# Autodesk Inventor assembly: Avionics
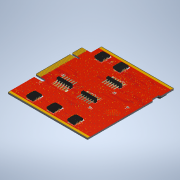
[picture p0: Inventor's stored thumbnail of the model, 180x180]
Saved by Autodesk Inventor 2021 (Build 250183000, 183)
## iProperties
Created: 2020-10-20
Part Number: Avionics
Document SubType Name: Assembly
Designer: Bradley
Author: Bradley
## Documents named in this file (35)
- C:\Users\Bradley\Documents\GitHub\CougSat1-Hardware\CougSat1-AvionicBoard\CADModel\Native\Avionics.iam
- C:\Users\Bradley\Documents\GitHub\CougSat1-Hardware\CougSat1-AvionicBoard\CADModel\Native\Avionics_PCB.ipt
- C:\Users\Bradley\Documents\GitHub\Resources\SupplierDocuments\04 - Connectors SMT\04-0001\04-0001.iam
- C:\Users\Bradley\Documents\GitHub\Resources\SupplierDocuments\04 - Connectors SMT\04-0008\04-0008.iam
- C:\Users\Bradley\Documents\GitHub\Resources\SupplierDocuments\21 - Resistor 1608\21-0000\21-0000.ipt
- C:\Users\Bradley\Documents\GitHub\Resources\SupplierDocuments\36 - Ferrite\36-152A\36-152A.ipt
- C:\Users\Bradley\Documents\GitHub\Resources\SupplierDocuments\11 - Capacitor Ceramic 1608\11-105A\11-105A.ipt
- C:\Users\Bradley\Documents\GitHub\Resources\SupplierDocuments\21 - Resistor 1608\21-1001\21-1001.ipt
- C:\Users\Bradley\Documents\GitHub\Resources\SupplierDocuments\16 - Capacitor Tantalum SMT\16-475A\16-475A.ipt
- C:\Users\Bradley\Documents\GitHub\Resources\SupplierDocuments\11 - Capacitor Ceramic 1608\11-682A\11-682A.ipt
- C:\Users\Bradley\Documents\GitHub\Resources\SupplierDocuments\40 - Crystal SMT\40-805A\40-805A.ipt
- C:\Users\Bradley\Documents\GitHub\Resources\SupplierDocuments\11 - Capacitor Ceramic 1608\11-106A\11-106A.ipt
- C:\Users\Bradley\Documents\GitHub\Resources\SupplierDocuments\21 - Resistor 1608\21-1002\21-1002.ipt
- C:\Users\Bradley\Documents\GitHub\Resources\SupplierDocuments\26 - Resistor Misc\26-0001\26-0001.ipt
- C:\Users\Bradley\Documents\GitHub\Resources\SupplierDocuments\26 - Resistor Misc\26-0008\26-0008.ipt
- C:\Users\Bradley\Documents\GitHub\Resources\SupplierDocuments\11 - Capacitor Ceramic 1608\11-103A\11-103A.ipt
- C:\Users\Bradley\Documents\GitHub\Resources\SupplierDocuments\11 - Capacitor Ceramic 1608\11-100A\11-100A.ipt
- C:\Users\Bradley\Documents\GitHub\Resources\SupplierDocuments\11 - Capacitor Ceramic 1608\11-150A\11-150A.ipt
- C:\Users\Bradley\Documents\GitHub\Resources\SupplierDocuments\26 - Resistor Misc\26-0006\26-0006.ipt
- C:\Users\Bradley\Documents\GitHub\Resources\SupplierDocuments\40 - Crystal SMT\40-323A\40-323A.ipt
- C:\Users\Bradley\Documents\GitHub\Resources\SupplierDocuments\31 - Inductor 1608\31-330A\31-330A.ipt
- C:\Users\Bradley\Documents\GitHub\Resources\SupplierDocuments\16 - Capacitor Tantalum SMT\16-476A\16-476A.ipt
- C:\Users\Bradley\Documents\GitHub\Resources\SupplierDocuments\21 - Resistor 1608\21-0.05\21-0.05.ipt
- C:\Users\Bradley\Documents\GitHub\Resources\SupplierDocuments\11 - Capacitor Ceramic 1608\11-104A\11-104A.ipt
- C:\Users\Bradley\Documents\GitHub\Resources\SupplierDocuments\27 - Conversion IC\27-0003\27-0003.ipt
- C:\Users\Bradley\Documents\GitHub\Resources\SupplierDocuments\08 - Amplifier (excluding RF)\08-0002\08-0002.ipt
- C:\Users\Bradley\Documents\GitHub\Resources\SupplierDocuments\63 - LED SMT\63-0004\63-0004.ipt
- C:\Users\Bradley\Documents\GitHub\Resources\SupplierDocuments\63 - LED SMT\63-0001\63-0001.ipt
- C:\Users\Bradley\Documents\GitHub\Resources\SupplierDocuments\04 - Connectors SMT\04-0005\04-0005.ipt
- C:\Users\Bradley\Documents\GitHub\Resources\SupplierDocuments\08 - Amplifier (excluding RF)\08-0004\08-0004.ipt
- C:\Users\Bradley\Documents\GitHub\Resources\SupplierDocuments\29 - Memory\29-0001\29-0001.ipt
- C:\Users\Bradley\Documents\GitHub\Resources\SupplierDocuments\61 - µController (and CLPD, FPGA,  etc.)\61-0002\61-0002.ipt
- C:\Users\Bradley\Documents\GitHub\Resources\SupplierDocuments\04 - Connectors SMT\04-0004\04-0004.ipt
- C:\Users\Bradley\Documents\GitHub\Resources\SupplierDocuments\09 - Communication IC\09-0001\09-0001.ipt
- C:\Users\Bradley\Documents\GitHub\Resources\SupplierDocuments\65 - RF\65-0001\65-0001.ipt
## Components (205 placed, 34 different names)
1. 65-0001:1 — Mate:483, Mate:484, Flush:131
2. 09-0001:8 — Mate:469, Mate:482, Flush:130
3. 09-0001:7 — Mate:470, Mate:481, Flush:129
4. 09-0001:6 — Mate:471, Mate:480, Flush:128
5. 09-0001:5 — Mate:472, Mate:479, Flush:127
6. 09-0001:4 — Mate:473, Flush:125, Flush:126
7. 09-0001:3 — Mate:474, Flush:123, Flush:124
8. 09-0001:2 — Mate:475, Flush:122, Mate:478
9. 09-0001:1 — Mate:476, Flush:121, Mate:477
10. 04-0004:3 — Mate:463, Mate:468, Flush:120
11. 04-0004:2 — Mate:464, Flush:119, Mate:467
12. 04-0004:1 — Mate:465, Flush:118, Mate:466
13. 61-0002:3 — Mate:461, Flush:117, Mate:462
14. 61-0002:2 — Mate:460, Flush:115, Flush:116
15. 61-0002:1 — Mate:459, Flush:113, Flush:114
16. 29-0001:2 — Mate:458, Flush:111, Flush:112
17. 29-0001:1 — Mate:457, Flush:109, Flush:110
18. 08-0004:3 — Mate:456, Flush:107, Flush:108
19. 08-0004:2 — Mate:455, Flush:105, Flush:106
20. 08-0004:1 — Mate:454, Flush:103, Flush:104
21. 04-0005:4 — Mate:442, Mate:452, Mate:453
22. 04-0005:3 — Mate:443, Mate:450, Mate:451
23. 04-0005:2 — Mate:444, Mate:448, Mate:449
24. 04-0005:1 — Mate:445, Mate:446, Mate:447
25. 63-0001:3 — Mate:438, Mate:441, Flush:102
26. 63-0001:2 — Mate:434, Mate:440, Flush:101
27. 63-0001:1 — Mate:433, Mate:439, Flush:100
28. 63-0004:1 — Mate:432, Mate:436, Mate:437
29. 08-0002:4 — Mate:429, Mate:431, Flush:99
30. 08-0002:3 — Mate:428, Mate:430, Flush:98
31. 08-0002:2 — Mate:427, Flush:96, Flush:97
32. 08-0002:1 — Mate:426, Flush:94, Flush:95
33. 27-0003:3 — Mate:423, Mate:425, Flush:93
34. 27-0003:2 — Mate:422, Flush:91, Flush:92
35. 27-0003:1 — Mate:421, Mate:424, Flush:90
36. 11-104A:59 — Mate:299, Mate:419, Mate:420
37. 11-104A:58 — Mate:301, Mate:417, Mate:418
38. 11-104A:57 — Mate:302, Mate:416, Flush:89
39. 11-104A:56 — Mate:305, Mate:415, Flush:88
40. 11-104A:55 — Mate:306, Mate:413, Mate:414
41. 11-104A:54 — Mate:309, Mate:411, Mate:412
42. 11-104A:53 — Mate:312, Mate:410, Flush:87
43. 11-104A:52 — Mate:313, Mate:409, Flush:86
44. 11-104A:51 — Mate:314, Mate:407, Mate:408
45. 11-104A:50 — Mate:317, Mate:405, Mate:406
46. 11-104A:49 — Mate:318, Mate:403, Mate:404
47. 11-104A:48 — Mate:322, Mate:401, Mate:402
48. 11-104A:47 — Mate:323, Mate:399, Mate:400
49. 11-104A:46 — Mate:324, Mate:398, Flush:85
50. 11-104A:45 — Mate:327, Mate:396, Mate:397
51. 11-104A:44 — Mate:328, Mate:394, Mate:395
52. 11-104A:43 — Mate:331, Mate:392, Mate:393
53. 11-104A:42 — Mate:294, Mate:391, Flush:84
54. 11-104A:41 — Mate:295, Mate:389, Mate:390
55. 11-104A:40 — Mate:296, Mate:388, Flush:83
56. 11-104A:39 — Mate:297, Mate:387, Flush:82
57. 11-104A:38 — Mate:298, Mate:386, Flush:81
58. 11-104A:37 — Mate:300, Mate:384, Mate:385
59. 11-104A:36 — Mate:303, Mate:383, Flush:80
60. 11-104A:35 — Mate:304, Mate:381, Mate:382
61. 11-104A:34 — Mate:307, Mate:380, Flush:79
62. 11-104A:33 — Mate:308, Mate:378, Mate:379
63. 11-104A:32 — Mate:310, Mate:377, Flush:78
64. 11-104A:31 — Mate:311, Mate:376, Flush:77
65. 11-104A:30 — Mate:315, Mate:375, Flush:76
66. 11-104A:29 — Mate:316, Mate:373, Mate:374
67. 11-104A:28 — Mate:319, Mate:372, Flush:75
68. 11-104A:27 — Mate:320, Mate:370, Mate:371
69. 11-104A:26 — Mate:321, Mate:369, Flush:74
70. 11-104A:25 — Mate:325, Mate:368, Flush:73
71. 11-104A:24 — Mate:326, Mate:367, Flush:72
72. 11-104A:23 — Mate:329, Mate:365, Mate:366
73. 11-104A:22 — Mate:330, Mate:364, Flush:71
74. 11-104A:21 — Mate:293, Mate:362, Mate:363
75. 11-104A:20 — Mate:291, Mate:360, Mate:361
76. 11-104A:19 — Mate:292, Mate:359, Flush:70
77. 11-104A:18 — Mate:290, Mate:358, Flush:69
78. 11-104A:17 — Mate:289, Mate:356, Mate:357
79. 11-104A:16 — Mate:288, Mate:355, Flush:68
80. 11-104A:15 — Mate:287, Mate:353, Mate:354
81. 11-104A:14 — Mate:286, Mate:351, Mate:352
82. 11-104A:13 — Mate:285, Mate:350, Flush:67
83. 11-104A:12 — Mate:284, Mate:349, Flush:66
84. 11-104A:11 — Mate:283, Mate:347, Mate:348
85. 11-104A:10 — Mate:282, Mate:346, Flush:65
86. 11-104A:9 — Mate:281, Mate:344, Mate:345
87. 11-104A:8 — Mate:280, Mate:343, Flush:64
88. 11-104A:7 — Mate:279, Mate:341, Mate:342
89. 11-104A:6 — Mate:278, Mate:340, Flush:63
90. 11-104A:5 — Mate:277, Mate:338, Mate:339
91. 11-104A:4 — Mate:276, Mate:336, Mate:337
92. 11-104A:3 — Mate:275, Mate:335, Flush:62
93. 11-104A:2 — Mate:274, Mate:334, Flush:61
94. 11-104A:1 — Mate:273, Mate:332, Mate:333
95. 21-0.05:3 — Mate:269, Mate:272, Flush:60
96. 21-0.05:2 — Mate:268, Mate:271, Flush:59
97. 21-0.05:1 — Mate:267, Mate:270, Flush:58
98. 16-476A:1 — Mate:264, Mate:265, Mate:266
99. 31-330A:1 — Mate:262, Mate:263, Flush:57
100. 40-323A:6 — Mate:251, Mate:260, Mate:261
101. 40-323A:5 — Mate:250, Mate:258, Mate:259
102. 40-323A:4 — Mate:249, Mate:256, Mate:257
103. 40-323A:3 — Mate:248, Mate:254, Mate:255
104. 40-323A:2 — Mate:247, Mate:253, Flush:56
105. 40-323A:1 — Mate:246, Mate:252, Flush:55
106. 26-0006:1 — Mate:243, Mate:244, Mate:245
107. 11-150A:12 — Mate:220, Mate:241, Mate:242
108. 11-150A:11 — Mate:219, Mate:239, Mate:240
109. 11-150A:10 — Mate:218, Mate:237, Mate:238
110. 11-150A:9 — Mate:217, Mate:235, Mate:236
111. 11-150A:8 — Mate:216, Mate:233, Mate:234
112. 11-150A:7 — Mate:215, Mate:231, Mate:232
113. 11-150A:6 — Mate:214, Mate:230, Flush:54
114. 11-150A:5 — Mate:213, Mate:229, Flush:53
115. 11-150A:4 — Mate:212, Mate:227, Mate:228
116. 11-150A:3 — Mate:211, Mate:225, Mate:226
117. 11-150A:2 — Mate:210, Mate:223, Mate:224
118. 11-150A:1 — Mate:209, Mate:221, Mate:222
119. 11-100A:6 — Mate:200, Mate:208, Flush:52
120. 11-100A:5 — Mate:199, Mate:206, Mate:207
121. 11-100A:4 — Mate:198, Mate:204, Mate:205
122. 11-100A:3 — Mate:197, Mate:203, Flush:51
123. 11-100A:2 — Mate:196, Mate:202, Flush:50
124. 11-100A:1 — Mate:195, Mate:201, Flush:49
125. 11-103A:3 — Mate:191, Mate:194, Flush:48
126. 11-103A:2 — Mate:190, Mate:193, Flush:47
127. 11-103A:1 — Mate:189, Mate:192, Flush:46
128. 26-0008:19 — Mate:160, Mate:187, Mate:188
129. 26-0008:18 — Mate:159, Mate:185, Mate:186
130. 26-0008:17 — Mate:158, Mate:184, Flush:45
131. 26-0008:16 — Mate:157, Mate:183, Flush:44
132. 26-0008:15 — Mate:156, Mate:181, Mate:182
133. 26-0008:14 — Mate:155, Mate:179, Mate:180
134. 26-0008:13 — Mate:154, Mate:178, Flush:43
135. 26-0008:12 — Mate:153, Mate:177, Flush:42
136. 26-0008:11 — Mate:152, Mate:175, Mate:176
137. 26-0008:10 — Mate:151, Mate:174, Flush:41
138. 26-0008:9 — Mate:150, Mate:173, Flush:40
139. 26-0008:8 — Mate:149, Mate:172, Flush:39
140. 26-0008:7 — Mate:148, Mate:171, Flush:38
141. 26-0008:6 — Mate:147, Mate:169, Mate:170
142. 26-0008:5 — Mate:146, Mate:167, Mate:168
143. 26-0008:4 — Mate:145, Mate:165, Mate:166
144. 26-0008:3 — Mate:144, Mate:163, Mate:164
145. 26-0008:2 — Mate:143, Mate:162, Flush:37
146. 26-0008:1 — Mate:142, Mate:161, Flush:36
147. 26-0001:3 — Mate:138, Mate:141, Flush:35
148. 26-0001:2 — Mate:137, Mate:140, Flush:34
149. 26-0001:1 — Mate:136, Mate:139, Flush:33
150. 21-1002:12 — Mate:116, Mate:133, Mate:134
151. 21-1002:11 — Mate:115, Mate:131, Mate:132
152. 21-1002:10 — Mate:114, Mate:130, Flush:31
153. 21-1002:9 — Mate:113, Mate:129, Flush:30
154. 21-1002:8 — Mate:112, Mate:128, Flush:29
155. 21-1002:7 — Mate:111, Mate:127, Flush:28
156. 21-1002:6 — Mate:110, Mate:126, Flush:27
157. 21-1002:5 — Mate:109, Mate:124, Mate:125
158. 21-1002:4 — Mate:108, Mate:123, Flush:26
159. 21-1002:3 — Mate:107, Mate:135, Flush:32
160. 21-1002:2 — Mate:106, Mate:119, Mate:120
161. 21-1002:1 — Mate:105, Mate:117, Mate:118
162. 11-106A:3 — Mate:98, Mate:103, Mate:104
163. 11-106A:2 — Mate:97, Mate:101, Mate:102
164. 11-106A:1 — Mate:96, Mate:99, Mate:100
165. 40-805A:3 — Mate:89, Mate:94, Mate:95
166. 40-805A:2 — Mate:90, Mate:93, Flush:25
167. 40-805A:1 — Mate:91, Mate:92, Flush:24
168. 11-682A:3 — Mate:85, Mate:88, Flush:23
169. 11-682A:2 — Mate:84, Mate:87, Flush:22
170. 11-682A:1 — Mate:83, Mate:86, Flush:21
171. 16-475A:2 — Mate:79, Mate:82, Flush:20
172. 16-475A:1 — Mate:78, Mate:80, Mate:81
173. 21-1001:11 — Mate:60, Mate:77, Flush:19
174. 21-1001:10 — Mate:59, Mate:76, Flush:18
175. 21-1001:9 — Mate:58, Mate:75, Flush:17
176. 21-1001:8 — Mate:57, Mate:73, Mate:74
177. 21-1001:7 — Mate:56, Mate:71, Mate:72
178. 21-1001:6 — Mate:55, Mate:69, Mate:70
179. 21-1001:5 — Mate:54, Mate:67, Mate:68
180. 21-1001:4 — Mate:53, Mate:65, Mate:66
181. 21-1001:3 — Mate:52, Mate:64, Flush:16
182. 21-1001:2 — Mate:51, Mate:62, Mate:63
183. 21-1001:1 — Mate:50, Mate:61, Flush:15
184. 11-105A:5 — Mate:41, Mate:48, Mate:49
185. 11-105A:4 — Mate:40, Mate:46, Mate:47
186. 11-105A:3 — Mate:39, Mate:44, Mate:45
187. 11-105A:2 — Mate:38, Mate:43, Flush:14
188. 11-105A:1 — Mate:37, Mate:42, Flush:13
189. 36-152A:2 — Mate:33, Mate:35, Mate:36
190. 36-152A:1 — Mate:32, Mate:34, Flush:12
191. 21-0000:7 — Mate:21, Mate:30, Mate:31
192. 21-0000:6 — Mate:20, Mate:29, Flush:11
193. 21-0000:5 — Mate:19, Mate:28, Flush:10
194. 21-0000:4 — Mate:18, Mate:26, Mate:27
195. 21-0000:3 — Mate:17, Mate:24, Mate:25
196. 21-0000:2 — Mate:16, Mate:23, Flush:9
197. 21-0000:1 — Mate:15, Mate:22, Flush:8
198. 04-0001:1 [sub-assembly] — Mate:1, Flush:1, Mate:8
199. 04-0001:2 [sub-assembly] — Mate:2, Flush:2, Mate:9
200. 04-0001:3 [sub-assembly] — Mate:3, Flush:3, Mate:10
201. 04-0001:4 [sub-assembly] — Mate:4, Flush:4, Mate:11
202. 04-0001:5 [sub-assembly] — Mate:5, Flush:5, Mate:12
203. 04-0001:6 [sub-assembly] — Mate:6, Flush:6, Mate:13
204. 04-0008:1 [sub-assembly] — Mate:7, Flush:7, Mate:14
205. Avionics_PCB:1 — Mate:1, Mate:2, Mate:3, Mate:4, Mate:5, Mate:6, Mate:7, Mate:15, Mate:16, Mate:17, Mate:18, Mate:19, Mate:20, Mate:21, Mate:32, Mate:33, Mate:37, Mate:38, Mate:39, Mate:40, Mate:41, Mate:50, Mate:51, Mate:52, Mate:53, Mate:54, Mate:55, Mate:56, Mate:57, Mate:58, Mate:59, Mate:60, Mate:78, Mate:79, Mate:83, Mate:84, Mate:85, Mate:89, Mate:90, Mate:91, Mate:96, Mate:97, Mate:98, Mate:105, Mate:106, Mate:107, Mate:108, Mate:109, Mate:110, Mate:111, Mate:112, Mate:113, Mate:114, Mate:115, Mate:116, Mate:136, Mate:137, Mate:138, Mate:142, Mate:143, Mate:144, Mate:145, Mate:146, Mate:147, Mate:148, Mate:149, Mate:150, Mate:151, Mate:152, Mate:153, Mate:154, Mate:155, Mate:156, Mate:157, Mate:158, Mate:159, Mate:160, Mate:189, Mate:190, Mate:191, Mate:195, Mate:196, Mate:197, Mate:198, Mate:199, Mate:200, Mate:209, Mate:210, Mate:211, Mate:212, Mate:213, Mate:214, Mate:215, Mate:216, Mate:217, Mate:218, Mate:219, Mate:220, Mate:243, Mate:246, Mate:247, Mate:248, Mate:249, Mate:250, Mate:251, Mate:262, Mate:264, Mate:267, Mate:268, Mate:269, Mate:273, Mate:274, Mate:275, Mate:276, Mate:277, Mate:278, Mate:279, Mate:280, Mate:281, Mate:282, Mate:283, Mate:284, Mate:285, Mate:286, Mate:287, Mate:288, Mate:289, Mate:290, Mate:291, Mate:292, Mate:293, Mate:294, Mate:295, Mate:296, Mate:297, Mate:298, Mate:299, Mate:300, Mate:301, Mate:302, Mate:303, Mate:304, Mate:305, Mate:306, Mate:307, Mate:308, Mate:309, Mate:310, Mate:311, Mate:312, Mate:313, Mate:314, Mate:315, Mate:316, Mate:317, Mate:318, Mate:319, Mate:320, Mate:321, Mate:322, Mate:323, Mate:324, Mate:325, Mate:326, Mate:327, Mate:328, Mate:329, Mate:330, Mate:331, Mate:421, Mate:422, Mate:423, Mate:426, Mate:427, Mate:428, Mate:429, Mate:432, Mate:433, Mate:434, Mate:438, Mate:442, Mate:443, Mate:444, Mate:445, Mate:454, Mate:455, Mate:456, Mate:457, Mate:458, Mate:459, Mate:460, Mate:461, Mate:463, Mate:464, Mate:465, Mate:469, Mate:470, Mate:471, Mate:472, Mate:473, Mate:474, Mate:475, Mate:476, Mate:483
## Relationships (612: Mate 481, Flush 131)
- Mate:1: 04-0001:1 ↔ Avionics_PCB:1
- Mate:2: 04-0001:2 ↔ Avionics_PCB:1
- Mate:3: 04-0001:3 ↔ Avionics_PCB:1
- Mate:4: 04-0001:4 ↔ Avionics_PCB:1
- Mate:5: 04-0001:5 ↔ Avionics_PCB:1
- Mate:6: 04-0001:6 ↔ Avionics_PCB:1
- Mate:7: 04-0008:1 ↔ Avionics_PCB:1
- Flush:1 (38 mm): 04-0001:1
- Flush:2 (38 mm): 04-0001:2
- Flush:3 (38 mm): 04-0001:3
- Flush:4 (-37.5 mm): 04-0001:4
- Flush:5 (-37.6 mm): 04-0001:5
- Mate:8 (25 mm): 04-0001:1
- Mate:9 (47.5 mm): 04-0001:2
- Mate:10 (70.5 mm): 04-0001:3
- Mate:11 (25 mm): 04-0001:4
- Mate:12 (45.5 mm): 04-0001:5
- Flush:6 (-84.2 mm): 04-0001:6
- Mate:13 (41 mm): 04-0001:6
- Flush:7 (12.1 mm): 04-0008:1
- Mate:14 (76.8 mm): 04-0008:1
- Mate:15: 21-0000:1 ↔ Avionics_PCB:1
- Mate:16: 21-0000:2 ↔ Avionics_PCB:1
- Mate:17: 21-0000:3 ↔ Avionics_PCB:1
- Mate:18: 21-0000:4 ↔ Avionics_PCB:1
- Mate:19: 21-0000:5 ↔ Avionics_PCB:1
- Mate:20: 21-0000:6 ↔ Avionics_PCB:1
- Mate:21: 21-0000:7 ↔ Avionics_PCB:1
- Mate:22 (9.5 mm): 21-0000:1
- Flush:8 (-12.5 mm): 21-0000:1
- Mate:23 (45 mm): 21-0000:2
- Flush:9 (-31.8 mm): 21-0000:2
- Mate:24 (-0.8 mm): 21-0000:3
- Mate:25 (54.4 mm): 21-0000:3
- Mate:26 (-6.5 mm): 21-0000:4
- Mate:27 (86.4 mm): 21-0000:4
- Mate:28 (34.2 mm): 21-0000:5
- Flush:10 (10.1 mm): 21-0000:5
- Mate:29 (52.4 mm): 21-0000:6
- Flush:11 (-30.8 mm): 21-0000:6
- Mate:30 (34.1 mm): 21-0000:7
- Mate:31 (26.8 mm): 21-0000:7
- Mate:32: 36-152A:1 ↔ Avionics_PCB:1
- Mate:33: 36-152A:2 ↔ Avionics_PCB:1
- Mate:34 (42.3 mm): 36-152A:1
- Flush:12 (-33.8 mm): 36-152A:1
- Mate:35 (15.9 mm): 36-152A:2
- Mate:36 (-19.3 mm): 36-152A:2
- Mate:37: 11-105A:1 ↔ Avionics_PCB:1
- Mate:38: 11-105A:2 ↔ Avionics_PCB:1
- Mate:39: 11-105A:3 ↔ Avionics_PCB:1
- Mate:40: 11-105A:4 ↔ Avionics_PCB:1
- Mate:41: 11-105A:5 ↔ Avionics_PCB:1
- Mate:42 (4.6 mm): 11-105A:1
- Flush:13 (-73.2 mm): 11-105A:1
- Mate:43 (-26.9 mm): 11-105A:2
- Flush:14 (-6.1 mm): 11-105A:2
- Mate:44 (8.6 mm): 11-105A:3
- Mate:45 (-29.3 mm): 11-105A:3
- Mate:46 (56.3 mm): 11-105A:4
- Mate:47 (32.7 mm): 11-105A:4
- Mate:48 (73.4 mm): 11-105A:5
- Mate:49 (32.8 mm): 11-105A:5
- Mate:50: 21-1001:1 ↔ Avionics_PCB:1
- Mate:51: 21-1001:2 ↔ Avionics_PCB:1
- Mate:52: 21-1001:3 ↔ Avionics_PCB:1
- Mate:53: 21-1001:4 ↔ Avionics_PCB:1
- Mate:54: 21-1001:5 ↔ Avionics_PCB:1
- Mate:55: 21-1001:6 ↔ Avionics_PCB:1
- Mate:56: 21-1001:7 ↔ Avionics_PCB:1
- Mate:57: 21-1001:8 ↔ Avionics_PCB:1
- Mate:58: 21-1001:9 ↔ Avionics_PCB:1
- Mate:59: 21-1001:10 ↔ Avionics_PCB:1
- Mate:60: 21-1001:11 ↔ Avionics_PCB:1
- Mate:61 (80.1 mm): 21-1001:1
- Flush:15 (-4 mm): 21-1001:1
- Mate:62 (17.6 mm): 21-1001:2
- Mate:63 (66.9 mm): 21-1001:2
- Mate:64 (67.5 mm): 21-1001:3
- Flush:16 (-19.9 mm): 21-1001:3
- Mate:65 (28.81 mm): 21-1001:4
- Mate:66 (56.41 mm): 21-1001:4
- Mate:67 (28.8 mm): 21-1001:5
- Mate:68 (54.7 mm): 21-1001:5
- Mate:69 (-1.99 mm): 21-1001:6
- Mate:70 (18.41 mm): 21-1001:6
- Mate:71 (25.3 mm): 21-1001:7
- Mate:72 (45.5 mm): 21-1001:7
- Mate:73 (-2.6 mm): 21-1001:8
- Mate:74 (45.6 mm): 21-1001:8
- Mate:75 (34.2 mm): 21-1001:9
- Flush:17 (14.7 mm): 21-1001:9
- Mate:76 (59 mm): 21-1001:10
- Flush:18 (-11.3 mm): 21-1001:10
- Mate:77 (59.1 mm): 21-1001:11
- Flush:19 (16.6 mm): 21-1001:11
- Mate:78: 16-475A:1 ↔ Avionics_PCB:1
- Mate:79: 16-475A:2 ↔ Avionics_PCB:1
- Mate:80 (40.2 mm): 16-475A:1
- Mate:81 (36.6 mm): 16-475A:1
- Mate:82 (13.7 mm): 16-475A:2
- Flush:20 (22.1 mm): 16-475A:2
- Mate:83: 11-682A:1 ↔ Avionics_PCB:1
- Mate:84: 11-682A:2 ↔ Avionics_PCB:1
- Mate:85: 11-682A:3 ↔ Avionics_PCB:1
- Mate:86 (27.3 mm): 11-682A:1
- Flush:21 (-35.6 mm): 11-682A:1
- Mate:87 (17.4 mm): 11-682A:2
- Flush:22 (-28.4 mm): 11-682A:2
- Mate:88 (27.2 mm): 11-682A:3
- Flush:23 (-17.9 mm): 11-682A:3
- Mate:89: 40-805A:3 ↔ Avionics_PCB:1
- Mate:90: 40-805A:2 ↔ Avionics_PCB:1
- Mate:91: 40-805A:1 ↔ Avionics_PCB:1
- Mate:92 (19.605 mm): 40-805A:1
- Flush:24 (-62.14 mm): 40-805A:1
- Mate:93 (-8.3 mm): 40-805A:2
- Flush:25 (-62.2 mm): 40-805A:2
- Mate:94 (27 mm): 40-805A:3
- Mate:95 (-17.8 mm): 40-805A:3
- Mate:96: 11-106A:1 ↔ Avionics_PCB:1
- Mate:97: 11-106A:2 ↔ Avionics_PCB:1
- Mate:98: 11-106A:3 ↔ Avionics_PCB:1
- Mate:99 (56.3 mm): 11-106A:1
- Mate:100 (37.3 mm): 11-106A:1
- Mate:101 (7.2 mm): 11-106A:2
- Mate:102 (-31 mm): 11-106A:2
- Mate:103 (73.4 mm): 11-106A:3
- Mate:104 (37.4 mm): 11-106A:3
- Mate:105: 21-1002:1 ↔ Avionics_PCB:1
- Mate:106: 21-1002:2 ↔ Avionics_PCB:1
- Mate:107: 21-1002:3 ↔ Avionics_PCB:1
- Mate:108: 21-1002:4 ↔ Avionics_PCB:1
- Mate:109: 21-1002:5 ↔ Avionics_PCB:1
- Mate:110: 21-1002:6 ↔ Avionics_PCB:1
- Mate:111: 21-1002:7 ↔ Avionics_PCB:1
- Mate:112: 21-1002:8 ↔ Avionics_PCB:1
- Mate:113: 21-1002:9 ↔ Avionics_PCB:1
- Mate:114: 21-1002:10 ↔ Avionics_PCB:1
- Mate:115: 21-1002:11 ↔ Avionics_PCB:1
- Mate:116: 21-1002:12 ↔ Avionics_PCB:1
- Mate:117 (4.6 mm): 21-1002:1
- Mate:118 (74.9 mm): 21-1002:1
- Mate:119 (36.1 mm): 21-1002:2
- Mate:120 (48.5 mm): 21-1002:2
- Mate:123 (23.3 mm): 21-1002:4
- Flush:26 (-31.2 mm): 21-1002:4
- Mate:124 (-20 mm): 21-1002:5
- Mate:125 (21.4 mm): 21-1002:5
- Mate:126 (41 mm): 21-1002:6
- Flush:27 (-31.2 mm): 21-1002:6
- Mate:127 (35 mm): 21-1002:7
- Flush:28 (-30.4 mm): 21-1002:7
- Mate:128 (33.8 mm): 21-1002:8
- Flush:29 (-21.3 mm): 21-1002:8
- Mate:129 (27.8 mm): 21-1002:9
- Flush:30 (-19.7 mm): 21-1002:9
- Mate:130 (17.3 mm): 21-1002:10
- Flush:31 (-29.5 mm): 21-1002:10
- Mate:131 (-20 mm): 21-1002:11
- Mate:132 (23.1 mm): 21-1002:11
- Mate:133 (36.1 mm): 21-1002:12
- Mate:134 (65.6 mm): 21-1002:12
- Mate:135 (9.3 mm): 21-1002:3
- Flush:32 (38.2 mm): 21-1002:3
- Mate:136: 26-0001:1 ↔ Avionics_PCB:1
- Mate:137: 26-0001:2 ↔ Avionics_PCB:1
- Mate:138: 26-0001:3 ↔ Avionics_PCB:1
- Mate:139 (52 mm): 26-0001:1
- Flush:33 (-40.7 mm): 26-0001:1
- Mate:140 (69.2 mm): 26-0001:2
- Flush:34 (-40.8 mm): 26-0001:2
- Mate:141 (6.6 mm): 26-0001:3
- Flush:35 (41.6 mm): 26-0001:3
- Mate:142: 26-0008:1 ↔ Avionics_PCB:1
- Mate:143: 26-0008:2 ↔ Avionics_PCB:1
- Mate:144: 26-0008:3 ↔ Avionics_PCB:1
- Mate:145: 26-0008:4 ↔ Avionics_PCB:1
- Mate:146: 26-0008:5 ↔ Avionics_PCB:1
- Mate:147: 26-0008:6 ↔ Avionics_PCB:1
- Mate:148: 26-0008:7 ↔ Avionics_PCB:1
- Mate:149: 26-0008:8 ↔ Avionics_PCB:1
- Mate:150: 26-0008:9 ↔ Avionics_PCB:1
- Mate:151: 26-0008:10 ↔ Avionics_PCB:1
- Mate:152: 26-0008:11 ↔ Avionics_PCB:1
- Mate:153: 26-0008:12 ↔ Avionics_PCB:1
- Mate:154: 26-0008:13 ↔ Avionics_PCB:1
- Mate:155: 26-0008:14 ↔ Avionics_PCB:1
- Mate:156: 26-0008:15 ↔ Avionics_PCB:1
- Mate:157: 26-0008:16 ↔ Avionics_PCB:1
- Mate:158: 26-0008:17 ↔ Avionics_PCB:1
- Mate:159: 26-0008:18 ↔ Avionics_PCB:1
- Mate:160: 26-0008:19 ↔ Avionics_PCB:1
- Mate:161 (-0.7 mm): 26-0008:1
- Flush:36 (-86.4 mm): 26-0008:1
- Mate:162 (15.6 mm): 26-0008:2
- Flush:37 (-88.9 mm): 26-0008:2
- Mate:163 (72.6 mm): 26-0008:3
- Mate:164 (29.3 mm): 26-0008:3
- Mate:165 (18.5 mm): 26-0008:4
- Mate:166 (38.2 mm): 26-0008:4
- Mate:167 (77.6 mm): 26-0008:5
- Mate:168 (-18.5 mm): 26-0008:5
- Mate:169 (34.8 mm): 26-0008:6
- Mate:170 (6.2 mm): 26-0008:6
- Mate:171 (27.1 mm): 26-0008:7
- Flush:38 (-60.6 mm): 26-0008:7
- Mate:172 (28 mm): 26-0008:8
- Flush:39 (-26 mm): 26-0008:8
- Mate:173 (28.9 mm): 26-0008:9
- Flush:40 (-43.6 mm): 26-0008:9
- Mate:174 (18 mm): 26-0008:10
- Flush:41 (-36.4 mm): 26-0008:10
- Mate:175 (67.1 mm): 26-0008:11
- Mate:176 (3.8 mm): 26-0008:11
- Mate:177 (-0.8 mm): 26-0008:12
- Flush:42 (-60.7 mm): 26-0008:12
- Mate:178 (-17.1 mm): 26-0008:13
- Flush:43 (-20.1 mm): 26-0008:13
- Mate:179 (23.5 mm): 26-0008:14
- Mate:180 (-24.3 mm): 26-0008:14
- Mate:181 (40.3 mm): 26-0008:15
- Mate:182 (-24.3 mm): 26-0008:15
- Mate:183 (15.6 mm): 26-0008:16
- Flush:44 (-83.3 mm): 26-0008:16
- Mate:184 (15.6 mm): 26-0008:17
- Flush:45 (-77.8 mm): 26-0008:17
- Mate:185 (57.6 mm): 26-0008:18
- Mate:186 (-24.3 mm): 26-0008:18
- Mate:187 (74.2 mm): 26-0008:19
- Mate:188 (-24.3 mm): 26-0008:19
- Mate:189: 11-103A:1 ↔ Avionics_PCB:1
- Mate:190: 11-103A:2 ↔ Avionics_PCB:1
- Mate:191: 11-103A:3 ↔ Avionics_PCB:1
- Mate:192 (-0.8 mm): 11-103A:1
- Flush:46 (-59 mm): 11-103A:1
- Mate:193 (-17.1 mm): 11-103A:2
- Flush:47 (-22.2 mm): 11-103A:2
- Mate:194 (27.1 mm): 11-103A:3
- Flush:48 (-58.9 mm): 11-103A:3
- Mate:195: 11-100A:1 ↔ Avionics_PCB:1
- Mate:196: 11-100A:2 ↔ Avionics_PCB:1
- Mate:197: 11-100A:3 ↔ Avionics_PCB:1
- Mate:198: 11-100A:4 ↔ Avionics_PCB:1
- Mate:199: 11-100A:5 ↔ Avionics_PCB:1
- Mate:200: 11-100A:6 ↔ Avionics_PCB:1
- Mate:201 (21.1 mm): 11-100A:1
- Flush:49 (-65.2 mm): 11-100A:1
- Mate:202 (-9.8 mm): 11-100A:2
- Flush:50 (-65.2 mm): 11-100A:2
- Mate:203 (18.1 mm): 11-100A:3
- Flush:51 (-65.2 mm): 11-100A:3
- Mate:204 (28.4 mm): 11-100A:4
- Mate:205 (-20.8 mm): 11-100A:4
- Mate:206 (25.5 mm): 11-100A:5
- Mate:207 (-20.8 mm): 11-100A:5
- Mate:208 (-6.9 mm): 11-100A:6
- Flush:52 (-65.2 mm): 11-100A:6
- Mate:209: 11-150A:1 ↔ Avionics_PCB:1
- Mate:210: 11-150A:2 ↔ Avionics_PCB:1
- Mate:211: 11-150A:3 ↔ Avionics_PCB:1
- Mate:212: 11-150A:4 ↔ Avionics_PCB:1
- Mate:213: 11-150A:5 ↔ Avionics_PCB:1
- Mate:214: 11-150A:6 ↔ Avionics_PCB:1
- Mate:215: 11-150A:7 ↔ Avionics_PCB:1
- Mate:216: 11-150A:8 ↔ Avionics_PCB:1
- Mate:217: 11-150A:9 ↔ Avionics_PCB:1
- Mate:218: 11-150A:10 ↔ Avionics_PCB:1
- Mate:219: 11-150A:11 ↔ Avionics_PCB:1
- Mate:220: 11-150A:12 ↔ Avionics_PCB:1
- Mate:221 (65.6 mm): 11-150A:1
- Mate:222 (26.1 mm): 11-150A:1
- Mate:223 (65.6 mm): 11-150A:2
- Mate:224 (23.7 mm): 11-150A:2
- Mate:225 (65.7 mm): 11-150A:3
- Mate:226 (-1.8 mm): 11-150A:3
- Mate:227 (65.7 mm): 11-150A:4
- Mate:228 (-4.2 mm): 11-150A:4
- Mate:229 (-19.8 mm): 11-150A:5
- Flush:53 (-33.5 mm): 11-150A:5
- Mate:230 (-19.8 mm): 11-150A:6
- Flush:54 (-31.1 mm): 11-150A:6
- Mate:231 (39.8 mm): 11-150A:7
- Mate:232 (21.9 mm): 11-150A:7
- Mate:233 (36.8 mm): 11-150A:8
- Mate:234 (21.9 mm): 11-150A:8
- Mate:235 (22.4 mm): 11-150A:9
- Mate:236 (21.9 mm): 11-150A:9
- Mate:237 (19.5 mm): 11-150A:10
- Mate:238 (21.9 mm): 11-150A:10
- Mate:239 (33 mm): 11-150A:11
- Mate:240 (12 mm): 11-150A:11
- Mate:241 (30.1 mm): 11-150A:12
- Mate:242 (12 mm): 11-150A:12
- Mate:243: 26-0006:1 ↔ Avionics_PCB:1
- Mate:244 (39 mm): 26-0006:1
- Mate:245 (61.2 mm): 26-0006:1
- Mate:246: 40-323A:1 ↔ Avionics_PCB:1
- Mate:247: 40-323A:2 ↔ Avionics_PCB:1
- Mate:248: 40-323A:3 ↔ Avionics_PCB:1
- Mate:249: 40-323A:4 ↔ Avionics_PCB:1
- Mate:250: 40-323A:5 ↔ Avionics_PCB:1
- Mate:251: 40-323A:6 ↔ Avionics_PCB:1
- Mate:252 (24.9 mm): 40-323A:1
- Flush:55 (-62.8 mm): 40-323A:1
- Mate:253 (-3 mm): 40-323A:2
- Flush:56 (-62.9 mm): 40-323A:2
- Mate:254 (32.3 mm): 40-323A:3
- Mate:255 (-17 mm): 40-323A:3
- Mate:256 (38.7 mm): 40-323A:4
- Mate:257 (24.1 mm): 40-323A:4
- Mate:258 (21 mm): 40-323A:5
- Mate:259 (24.1 mm): 40-323A:5
- Mate:260 (31.5 mm): 40-323A:6
- Mate:261 (14.2 mm): 40-323A:6
- Mate:262: 31-330A:1 ↔ Avionics_PCB:1
- Mate:263 (76 mm): 31-330A:1
- Flush:57 (8.8 mm): 31-330A:1
- Mate:264: 16-476A:1 ↔ Avionics_PCB:1
- Mate:265 (15.9 mm): 16-476A:1
- Mate:266 (71.8 mm): 16-476A:1
- Mate:267: 21-0.05:1 ↔ Avionics_PCB:1
- Mate:268: 21-0.05:2 ↔ Avionics_PCB:1
- Mate:269: 21-0.05:3 ↔ Avionics_PCB:1
- Mate:270 (80.3 mm): 21-0.05:1
- Flush:58 (-19.9 mm): 21-0.05:1
- Mate:271 (74.9 mm): 21-0.05:2
- Flush:59 (-19.9 mm): 21-0.05:2
- Mate:272 (86 mm): 21-0.05:3
- Flush:60 (-19.9 mm): 21-0.05:3
- Mate:273: 11-104A:1 ↔ Avionics_PCB:1
- Mate:274: 11-104A:2 ↔ Avionics_PCB:1
- Mate:275: 11-104A:3 ↔ Avionics_PCB:1
- Mate:276: 11-104A:4 ↔ Avionics_PCB:1
- Mate:277: 11-104A:5 ↔ Avionics_PCB:1
- Mate:278: 11-104A:6 ↔ Avionics_PCB:1
- Mate:279: 11-104A:7 ↔ Avionics_PCB:1
- Mate:280: 11-104A:8 ↔ Avionics_PCB:1
- Mate:281: 11-104A:9 ↔ Avionics_PCB:1
- Mate:282: 11-104A:10 ↔ Avionics_PCB:1
- Mate:283: 11-104A:11 ↔ Avionics_PCB:1
- Mate:284: 11-104A:12 ↔ Avionics_PCB:1
- Mate:285: 11-104A:13 ↔ Avionics_PCB:1
- Mate:286: 11-104A:14 ↔ Avionics_PCB:1
- Mate:287: 11-104A:15 ↔ Avionics_PCB:1
- Mate:288: 11-104A:16 ↔ Avionics_PCB:1
- Mate:289: 11-104A:17 ↔ Avionics_PCB:1
- Mate:290: 11-104A:18 ↔ Avionics_PCB:1
- Mate:291: 11-104A:20 ↔ Avionics_PCB:1
- Mate:292: 11-104A:19 ↔ Avionics_PCB:1
- Mate:293: 11-104A:21 ↔ Avionics_PCB:1
- Mate:294: 11-104A:42 ↔ Avionics_PCB:1
- Mate:295: 11-104A:41 ↔ Avionics_PCB:1
- Mate:296: 11-104A:40 ↔ Avionics_PCB:1
- Mate:297: 11-104A:39 ↔ Avionics_PCB:1
- Mate:298: 11-104A:38 ↔ Avionics_PCB:1
- Mate:299: 11-104A:59 ↔ Avionics_PCB:1
- Mate:300: 11-104A:37 ↔ Avionics_PCB:1
- Mate:301: 11-104A:58 ↔ Avionics_PCB:1
- Mate:302: 11-104A:57 ↔ Avionics_PCB:1
- Mate:303: 11-104A:36 ↔ Avionics_PCB:1
- Mate:304: 11-104A:35 ↔ Avionics_PCB:1
- Mate:305: 11-104A:56 ↔ Avionics_PCB:1
- Mate:306: 11-104A:55 ↔ Avionics_PCB:1
- Mate:307: 11-104A:34 ↔ Avionics_PCB:1
- Mate:308: 11-104A:33 ↔ Avionics_PCB:1
- Mate:309: 11-104A:54 ↔ Avionics_PCB:1
- Mate:310: 11-104A:32 ↔ Avionics_PCB:1
- Mate:311: 11-104A:31 ↔ Avionics_PCB:1
- Mate:312: 11-104A:53 ↔ Avionics_PCB:1
- Mate:313: 11-104A:52 ↔ Avionics_PCB:1
- Mate:314: 11-104A:51 ↔ Avionics_PCB:1
- Mate:315: 11-104A:30 ↔ Avionics_PCB:1
- Mate:316: 11-104A:29 ↔ Avionics_PCB:1
- Mate:317: 11-104A:50 ↔ Avionics_PCB:1
- Mate:318: 11-104A:49 ↔ Avionics_PCB:1
- Mate:319: 11-104A:28 ↔ Avionics_PCB:1
- Mate:320: 11-104A:27 ↔ Avionics_PCB:1
- Mate:321: 11-104A:26 ↔ Avionics_PCB:1
- Mate:322: 11-104A:48 ↔ Avionics_PCB:1
- Mate:323: 11-104A:47 ↔ Avionics_PCB:1
- Mate:324: 11-104A:46 ↔ Avionics_PCB:1
- Mate:325: 11-104A:25 ↔ Avionics_PCB:1
- Mate:326: 11-104A:24 ↔ Avionics_PCB:1
- Mate:327: 11-104A:45 ↔ Avionics_PCB:1
- Mate:328: 11-104A:44 ↔ Avionics_PCB:1
- Mate:329: 11-104A:23 ↔ Avionics_PCB:1
- Mate:330: 11-104A:22 ↔ Avionics_PCB:1
- Mate:331: 11-104A:43 ↔ Avionics_PCB:1
- Mate:332 (77.2 mm): 11-104A:1
- Mate:333 (4 mm): 11-104A:1
- Mate:334 (-3.6 mm): 11-104A:2
- Flush:61 (-86.4 mm): 11-104A:2
- Mate:335 (-37.1 mm): 11-104A:3
- Flush:62 (-12 mm): 11-104A:3
- Mate:336 (49.5 mm): 11-104A:4
- Mate:337 (26.5 mm): 11-104A:4
- Mate:338 (52.4 mm): 11-104A:5
- Mate:339 (29 mm): 11-104A:5
- Mate:340 (-38 mm): 11-104A:6
- Flush:63 (-29.2 mm): 11-104A:6
- Mate:341 (30.9 mm): 11-104A:7
- Mate:342 (21.3 mm): 11-104A:7
- Mate:343 (24.4 mm): 11-104A:8
- Flush:64 (-35.5 mm): 11-104A:8
- Mate:344 (38.1 mm): 11-104A:9
- Mate:345 (31.2 mm): 11-104A:9
- Mate:346 (14.5 mm): 11-104A:10
- Flush:65 (-28.4 mm): 11-104A:10
- Mate:347 (20.4 mm): 11-104A:11
- Mate:348 (31.2 mm): 11-104A:11
- Mate:349 (27.2 mm): 11-104A:12
- Flush:66 (-16.2 mm): 11-104A:12
- Mate:350 (17.4 mm): 11-104A:13
- Flush:67 (-26.7 mm): 11-104A:13
- Mate:351 (56.1 mm): 11-104A:14
- Mate:352 (11.3 mm): 11-104A:14
- Mate:353 (49.6 mm): 11-104A:15
- Mate:354 (11.3 mm): 11-104A:15
- Mate:355 (22.4 mm): 11-104A:16
- Flush:68 (-45.5 mm): 11-104A:16
- Mate:356 (56.6 mm): 11-104A:17
- Mate:357 (26.5 mm): 11-104A:17
- Mate:358 (24.2 mm): 11-104A:18
- Flush:69 (-17.895 mm): 11-104A:18
- Mate:359 (35.1 mm): 11-104A:19
- Flush:70 (-72.8 mm): 11-104A:19
- Mate:360 (56.2 mm): 11-104A:20
- Mate:361 (-16.6 mm): 11-104A:20
- Mate:362 (49.7 mm): 11-104A:21
- Mate:363 (-16.6 mm): 11-104A:21
- Mate:364 (-5.5 mm): 11-104A:22
- Flush:71 (-45.6 mm): 11-104A:22
- Mate:365 (56.7 mm): 11-104A:23
- Mate:366 (-1.4 mm): 11-104A:23
- Mate:367 (27.3 mm): 11-104A:24
- Flush:72 (-33.9 mm): 11-104A:24
- Mate:368 (-12.2 mm): 11-104A:25
- Flush:73 (-18.4 mm): 11-104A:25
- Mate:369 (-4.9 mm): 11-104A:26
- Flush:74 (-18.4 mm): 11-104A:26
- Mate:370 (29.5 mm): 11-104A:27
- Mate:371 (-1.3 mm): 11-104A:27
- Mate:372 (-12.4 mm): 11-104A:28
- Flush:75 (-33.6 mm): 11-104A:28
- Mate:373 (10.2 mm): 11-104A:29
- Mate:374 (-31 mm): 11-104A:29
- Mate:375 (-26.9 mm): 11-104A:30
- Flush:76 (-4.4 mm): 11-104A:30
- Mate:376 (35 mm): 11-104A:31
- Flush:77 (-55.7 mm): 11-104A:31
- Mate:377 (12.2 mm): 11-104A:32
- Flush:78 (-80.1 mm): 11-104A:32
- Mate:378 (80.9 mm): 11-104A:33
- Mate:379 (18.2 mm): 11-104A:33
- Mate:380 (12.2 mm): 11-104A:34
- Flush:79 (-74.6 mm): 11-104A:34
- Mate:381 (75.4 mm): 11-104A:35
- Mate:382 (18.2 mm): 11-104A:35
- Mate:383 (12.2 mm): 11-104A:36
- Flush:80 (-85.7 mm): 11-104A:36
- Mate:384 (86.5 mm): 11-104A:37
- Mate:385 (18.2 mm): 11-104A:37
- Mate:386 (33.2 mm): 11-104A:38
- Flush:81 (-48.5 mm): 11-104A:38
- Mate:387 (35 mm): 11-104A:39
- Flush:82 (-57.4 mm): 11-104A:39
- Mate:388 (33.2 mm): 11-104A:40
- Flush:83 (-65.6 mm): 11-104A:40
- Mate:389 (75.1 mm): 11-104A:41
- Mate:390 (43.8 mm): 11-104A:41
- Mate:391 (-38 mm): 11-104A:42
- Flush:84 (-46.1 mm): 11-104A:42
- Mate:392 (80.2 mm): 11-104A:43
- Mate:393 (24.9 mm): 11-104A:43
- Mate:394 (74.9 mm): 11-104A:44
- Mate:395 (24.9 mm): 11-104A:44
- Mate:396 (86 mm): 11-104A:45
- Mate:397 (24.9 mm): 11-104A:45
- Mate:398 (39.4 mm): 11-104A:46
- Flush:85 (-33.8 mm): 11-104A:46
- Mate:399 (13 mm): 11-104A:47
- Mate:400 (-19.3 mm): 11-104A:47
- Mate:401 (22.7 mm): 11-104A:48
- Mate:402 (9 mm): 11-104A:48
- Mate:403 (22.7 mm): 11-104A:49
- Mate:404 (3.1 mm): 11-104A:49
- Mate:405 (50.7 mm): 11-104A:50
- Mate:406 (9.6 mm): 11-104A:50
- Mate:407 (47.8 mm): 11-104A:51
- Mate:408 (7.1 mm): 11-104A:51
- Mate:409 (-38.6 mm): 11-104A:52
- Flush:86 (-63 mm): 11-104A:52
- Mate:410 (-39.4 mm): 11-104A:53
- Flush:87 (-79.9 mm): 11-104A:53
- Mate:411 (52.1 mm): 11-104A:54
- Mate:412 (-20.8 mm): 11-104A:54
- Mate:413 (55 mm): 11-104A:55
- Mate:414 (-18.4 mm): 11-104A:55
- Mate:415 (-2.1 mm): 11-104A:56
- Flush:88 (-34.1 mm): 11-104A:56
- Mate:416 (-5 mm): 11-104A:57
- Flush:89 (-36.5 mm): 11-104A:57
- Mate:417 (57.9 mm): 11-104A:58
- Mate:418 (43.7 mm): 11-104A:58
- Mate:419 (11.5 mm): 11-104A:59
- Mate:420 (-29.3 mm): 11-104A:59
- Mate:421: 27-0003:1 ↔ Avionics_PCB:1
- Mate:422: 27-0003:2 ↔ Avionics_PCB:1
- Mate:423: 27-0003:3 ↔ Avionics_PCB:1
- Mate:424 (35.1 mm): 27-0003:1
- Flush:90 (-69.2 mm): 27-0003:1
- Flush:91 (-8.4 mm): 27-0003:2
- Flush:92 (34.6 mm): 27-0003:2
- Mate:425 (35 mm): 27-0003:3
- Flush:93 (-52.1 mm): 27-0003:3
- Mate:426: 08-0002:1 ↔ Avionics_PCB:1
- Mate:427: 08-0002:2 ↔ Avionics_PCB:1
- Mate:428: 08-0002:3 ↔ Avionics_PCB:1
- Mate:429: 08-0002:4 ↔ Avionics_PCB:1
- Flush:94 (-57.7 mm): 08-0002:1
- Flush:95 (-40.5 mm): 08-0002:1
- Flush:96 (-74.9 mm): 08-0002:2
- Flush:97 (-40.6 mm): 08-0002:2
- Mate:430 (35.5 mm): 08-0002:3
- Flush:98 (-60.6 mm): 08-0002:3
- Mate:431 (-26.4 mm): 08-0002:4
- Flush:99 (-9.3 mm): 08-0002:4
- Mate:432: 63-0004:1 ↔ Avionics_PCB:1
- Mate:433: 63-0001:1 ↔ Avionics_PCB:1
- Mate:434: 63-0001:2 ↔ Avionics_PCB:1
- Mate:436 (83.2 mm): 63-0004:1
- Mate:437 (4 mm): 63-0004:1
- Mate:438: 63-0001:3 ↔ Avionics_PCB:1
- Mate:439 (-17.3 mm): 63-0001:1
- Flush:100 (-62.1 mm): 63-0001:1
- Mate:440 (10.4 mm): 63-0001:2
- Flush:101 (-62 mm): 63-0001:2
- Mate:441 (-0.9 mm): 63-0001:3
- Flush:102 (-16.7 mm): 63-0001:3
- Mate:442: 04-0005:4 ↔ Avionics_PCB:1
- Mate:443: 04-0005:3 ↔ Avionics_PCB:1
- Mate:444: 04-0005:2 ↔ Avionics_PCB:1
- Mate:445: 04-0005:1 ↔ Avionics_PCB:1
- Mate:446 (47.4 mm): 04-0005:1
- Mate:447 (-41.5 mm): 04-0005:1
- Mate:448 (64.3 mm): 04-0005:2
- Mate:449 (-41.5 mm): 04-0005:2
- Mate:450 (13.6 mm): 04-0005:3
- Mate:451 (-41.5 mm): 04-0005:3
- Mate:452 (30.5 mm): 04-0005:4
- Mate:453 (-41.5 mm): 04-0005:4
- Mate:454: 08-0004:1 ↔ Avionics_PCB:1
- Mate:455: 08-0004:2 ↔ Avionics_PCB:1
- Mate:456: 08-0004:3 ↔ Avionics_PCB:1
- Flush:103 (-79.9 mm): 08-0004:1
- Flush:104 (-22.4 mm): 08-0004:1
- Flush:105 (-74.6 mm): 08-0004:2
- Flush:106 (-22.4 mm): 08-0004:2
- Flush:107 (-85.7 mm): 08-0004:3
- Flush:108 (-22.4 mm): 08-0004:3
- Mate:457: 29-0001:1 ↔ Avionics_PCB:1
- Mate:458: 29-0001:2 ↔ Avionics_PCB:1
- Flush:109 (-17.3 mm): 29-0001:1
- Flush:110 (-10.9 mm): 29-0001:1
- Flush:111 (-17.3 mm): 29-0001:2
- Flush:112 (-5 mm): 29-0001:2
- Mate:459: 61-0002:1 ↔ Avionics_PCB:1
- Mate:460: 61-0002:2 ↔ Avionics_PCB:1
- Mate:461: 61-0002:3 ↔ Avionics_PCB:1
- Flush:113 (9 mm): 61-0002:1
- Flush:114 (-53.2 mm): 61-0002:1
- Flush:115 (-18.9 mm): 61-0002:2
- Flush:116 (-53.1 mm): 61-0002:2
- Flush:117 (-26 mm): 61-0002:3
- Mate:462 (-8.9 mm): 61-0002:3
- Mate:463: 04-0004:3 ↔ Avionics_PCB:1
- Mate:464: 04-0004:2 ↔ Avionics_PCB:1
- Mate:465: 04-0004:1 ↔ Avionics_PCB:1
- Flush:118 (-46.75 mm): 04-0004:1
- Mate:466 (18.9 mm): 04-0004:1
- Flush:119 (-46.85 mm): 04-0004:2
- Mate:467 (-9 mm): 04-0004:2
- Mate:468 (32.35 mm): 04-0004:3
- Flush:120 (8.9 mm): 04-0004:3
- Mate:469: 09-0001:8 ↔ Avionics_PCB:1
- Mate:470: 09-0001:7 ↔ Avionics_PCB:1
- Mate:471: 09-0001:6 ↔ Avionics_PCB:1
- Mate:472: 09-0001:5 ↔ Avionics_PCB:1
- Mate:473: 09-0001:4 ↔ Avionics_PCB:1
- Mate:474: 09-0001:3 ↔ Avionics_PCB:1
- Mate:475: 09-0001:2 ↔ Avionics_PCB:1
- Mate:476: 09-0001:1 ↔ Avionics_PCB:1
- Flush:121 (-28.6 mm): 09-0001:1
- Mate:477 (49.5 mm): 09-0001:1
- Flush:122 (-26.9 mm): 09-0001:2
- Mate:478 (52.4 mm): 09-0001:2
- Flush:123 (-34.4 mm): 09-0001:3
- Flush:124 (5 mm): 09-0001:3
- Flush:125 (-36.2 mm): 09-0001:4
- Flush:126 (2.1 mm): 09-0001:4
- Mate:479 (7.5 mm): 09-0001:5
- Flush:127 (-50.7 mm): 09-0001:5
- Mate:480 (9.2 mm): 09-0001:6
- Flush:128 (-47.8 mm): 09-0001:6
- Mate:481 (-20.5 mm): 09-0001:7
- Flush:129 (-55 mm): 09-0001:7
- Mate:482 (-18.7 mm): 09-0001:8
- Flush:130 (-52.1 mm): 09-0001:8
- Mate:483: 65-0001:1 ↔ Avionics_PCB:1
- Mate:484 (-2.4 mm): 65-0001:1
- Flush:131 (-80 mm): 65-0001:1
